# Autodesk Inventor assembly: Assembly1
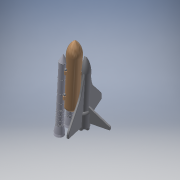
[picture p0: Inventor's stored thumbnail of the model, 180x180]
Saved by Autodesk Inventor 2018 (Build 220112000, 112)
## iProperties
Created: 2020-03-10
Part Number: Assembly1
Document SubType Name: Assembly
Designer: student
Author: student
## Documents named in this file (4)
- C:\alphamegazord\drive-download-20200310T233116Z-001\Assembly1.iam
- C:\alphamegazord\drive-download-20200310T233116Z-001\booster(2 of same model)_space shuttle.ipt
- C:\alphamegazord\drive-download-20200310T233116Z-001\orbiter_space shuttle.ipt
- C:\alphamegazord\drive-download-20200310T233116Z-001\tank_space shuttle.ipt
## Components (4 placed, 3 different names)
1. booster(2 of same model)_space shuttle:1 — Rigid:1
2. orbiter_space shuttle:1 — Rigid:2
3. tank_space shuttle:1 — Rigid:1, Cylindrical:1, Rigid:2
4. booster(2 of same model)_space shuttle:2 — Cylindrical:1
## Relationships (3: WeldJoint 2, CylindricalJoint 1)
- Rigid:1 [WeldJoint]: booster(2 of same model)_space shuttle:1 ↔ tank_space shuttle:1
- Cylindrical:1: tank_space shuttle:1 ↔ booster(2 of same model)_space shuttle:2
- Rigid:2 [WeldJoint]: orbiter_space shuttle:1 ↔ tank_space shuttle:1
